# Autodesk Inventor assembly: 足全体
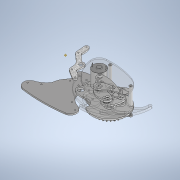
[picture p0: Inventor's stored thumbnail of the model, 180x180]
Saved by Autodesk Inventor 2022.2 (Build 262287030, 287C)
## iProperties
Created: 2022-01-30
Part Number: 足全体
Document SubType Name: Assembly
Designer: acps
Author: acps
## Documents named in this file (4)
- C:\Users\acps\Documents\srdc\srdc_ksh\足全体.iam
- C:\Users\acps\Documents\srdc\srdc_ksh\中間ユニット外.ipt
- C:\Users\acps\Documents\srdc\srdc_ksh\アーノン.ipt
- C:\Users\acps\Documents\srdc\srdc_ksh\足ユニット.iam
## Components (3 placed, 3 different names)
1. 中間ユニット外:1 — Mate:1, Mate:2
2. アーノン:1 — Mate:1, Mate:2, Mate:3
3. 足ユニット:1 [sub-assembly] — Mate:3
## Relationships (3: Mate 3)
- Mate:1: 中間ユニット外:1 ↔ アーノン:1
- Mate:2: 中間ユニット外:1 ↔ アーノン:1
- Mate:3: アーノン:1 ↔ 足ユニット:1
